# Autodesk Inventor assembly: mesoSPIM_excitation_path
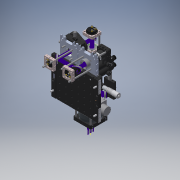
[picture p0: Inventor's stored thumbnail of the model, 180x180]
Saved by Autodesk Inventor 2016 (Build 200138000, 138)
## iProperties
Created: 2018-08-27
Part Number: mesoSPIM_excitation_path
Document SubType Name: Assembly
Designer: voigt
Author: voigt
## Documents named in this file (41)
- D:\Microscope_Design\CAD_Files\mesoSPIM_design_V5\mesoSPIM\excitation_path\mesoSPIM_excitation_path.iam
- D:\Microscope_Design\CAD_Files\mesoSPIM_design_V5\library\Thorlabs\large_area_translation_stages\tbb1515\TBB1515_M-Step.ipt
- D:\Microscope_Design\CAD_Files\mesoSPIM_design_V5\mesoSPIM\excitation_path\components\Galvomount-22mm-diameter-Thorlabs-Right.ipt
- D:\Microscope_Design\CAD_Files\mesoSPIM_design_V5\library\Thorlabs\posts\1_inch_posts\RS2P_M.ipt
- D:\Microscope_Design\CAD_Files\mesoSPIM_design_V5\library\Thorlabs\posts\1_5_inch_post_spacers\PS5M.ipt
- D:\Microscope_Design\CAD_Files\mesoSPIM_design_V5\library\Qioptiq\FLS40_rails\FLS40_150mm.ipt
- D:\Microscope_Design\CAD_Files\mesoSPIM_design_V5\library\Thorlabs\30mm_cage_system\base_plates\CPVM-60mm_Baseplate.ipt
- D:\Microscope_Design\CAD_Files\mesoSPIM_design_V5\library\Thorlabs\optics\AC254-075-A-ML-Step.ipt
- D:\Microscope_Design\CAD_Files\mesoSPIM_design_V5\mesoSPIM\optical_design\cad_export_v1\mesoSPIM_excitation_path_optics_V1.iam
- D:\Microscope_Design\CAD_Files\mesoSPIM_design_V5\library\Qioptiq\FLS40_carriers\FLS40_40mm_carrier.ipt
- D:\Microscope_Design\CAD_Files\mesoSPIM_design_V5\library\Qioptiq\microbench\Cube_30_with35hole.ipt
- D:\Microscope_Design\CAD_Files\mesoSPIM_design_V5\library\Qioptiq\microbench\Mounting_Plate_30.ipt
- D:\Microscope_Design\CAD_Files\mesoSPIM_design_V5\mesoSPIM\excitation_path\components\fold_mirror.iam
- D:\Microscope_Design\CAD_Files\mesoSPIM_design_V5\library\Qioptiq\FLS40_carriers\FLS40_20mm_carrier.ipt
- D:\Microscope_Design\CAD_Files\mesoSPIM_design_V5\library\Qioptiq\microbench\Mounting_Plate_35.ipt
- D:\Microscope_Design\CAD_Files\mesoSPIM_design_V5\library\Thorlabs\30mm_cage_system\cage_rods\ER3_CageRod.ipt
- D:\Microscope_Design\CAD_Files\Library_Files\Thorlabs\30mm_cage_system\rods\ER_CageRod.ipt
- D:\Microscope_Design\CAD_Files\mesoSPIM_design_V5\library\Thorlabs\30mm_cage_system\xy_mount\ST1XY-S_M-Step.ipt
- D:\Microscope_Design\CAD_Files\mesoSPIM_design_V5\library\Thorlabs\accessoires\SM1A39_Adapter_CmountExternal_SM1_External.ipt
- D:\Microscope_Design\CAD_Files\mesoSPIM_design_V5\library\Optotune\EL-16-40\EL-16-40-TC-C (133-193-03-R0-01).iam
- D:\Microscope_Design\CAD_Files\mesoSPIM_design_V5\library\Thorlabs\30mm_cage_system\cage_rods\ER1_CageRod.ipt
- D:\Microscope_Design\CAD_Files\mesoSPIM_design_V5\library\Thorlabs\30mm_cage_system\cage_rods\ER4_CageRod.ipt
- D:\Microscope_Design\CAD_Files\mesoSPIM_design_V5\library\Thorlabs\30mm_cage_system\cage_rods\ER2_CageRod.ipt
- D:\Microscope_Design\CAD_Files\mesoSPIM_design_V5\mesoSPIM\excitation_path\components\60mm-blank-cageplate-LCP03M-Nikon-MOD.ipt
- D:\Microscope_Design\CAD_Files\mesoSPIM_design_V5\library\Thorlabs\other\F-Mount-AdapterSM2NFM-Step.ipt
- D:\Microscope_Design\CAD_Files\mesoSPIM_design_V5\library\Nikon\50mm_1_4G_body_disassembled.ipt
- D:\Microscope_Design\CAD_Files\mesoSPIM_design_V5\library\Thorlabs\accessoires\SM1FCA-APC-Fiberadapter.ipt
- D:\Microscope_Design\CAD_Files\mesoSPIM_design_V5\library\Thorlabs\30mm_cage_system\cage_plates\SHCP025-Quarter-Inch-Shutter-Mount.ipt
- D:\Microscope_Design\CAD_Files\mesoSPIM_design_V5\library\Thorlabs\30mm_cage_system\cage_plates\CP02_M.ipt
- D:\Microscope_Design\CAD_Files\mesoSPIM_design_V5\library\Thorlabs\shutters\SHB025-Shutter.ipt
- D:\Microscope_Design\CAD_Files\mesoSPIM_design_V5\library\Thorlabs\30mm_cage_system\SM1_tubes\SM1L10.ipt
- D:\Microscope_Design\CAD_Files\mesoSPIM_design_V5\library\Thorlabs\30mm_cage_system\SM1_tubes\SM1V10.ipt
- D:\Microscope_Design\CAD_Files\mesoSPIM_design_V5\library\Qioptiq\microbench\35mm_lens_mount\35mm Lens Mount.ipt
- D:\Microscope_Design\CAD_Files\mesoSPIM_design_V5\library\Thorlabs\stages\XRN-B1_M-Micrometer-Baseplate.ipt
- D:\Microscope_Design\CAD_Files\mesoSPIM_design_V5\library\Thorlabs\stages\XRN25C_M-25mm-Micrometer-Stage-Simplified.ipt
- D:\Microscope_Design\CAD_Files\mesoSPIM_design_V5\library\Thorlabs\posts\post_mounts\PH75_M-Step.ipt
- D:\Microscope_Design\CAD_Files\mesoSPIM_design_V5\library\Thorlabs\posts\12_7_mm_posts\TR50M.ipt
- D:\Microscope_Design\CAD_Files\mesoSPIM_design_V5\library\Thorlabs\posts\12_7_mm_post_accessoires\RA180_M.ipt
- D:\Microscope_Design\CAD_Files\mesoSPIM_design_V5\library\Qioptiq\microbench\Microbench_Holder_30.iam
- D:\Microscope_Design\CAD_Files\mesoSPIM_design_V5\library\Thorlabs\posts\12_7_mm_posts\TR75M.ipt
- D:\Microscope_Design\CAD_Files\mesoSPIM_design_V5\library\Thorlabs\galvos\GVS411_M.ipt
## Components (62 placed, 39 different names)
1. TBB1515_M-Step:1 — Flush:1, Mate:1, Mate:2, Mate:3, Mate:4, Mate:5, Mate:6, Mate:7, Mate:8, Mate:10, Mate:18, Mate:19, Mate:20, Mate:22, Mate:96, Mate:97, Mate:98
2. Galvomount-22mm-diameter-Thorlabs-Right:1 — Mate:4, Mate:5, Mate:6, Flush:3, Mate:24, Mate:31, Mate:71, Mate:72, Flush:24, Angle:6, Mate:78, Angle:7, Mate:117, Mate:118, Angle:9
3. RS2P_M:1 — Mate:7, Mate:10, Mate:11, Mate:12
4. RS2P_M:2 — Mate:8, Mate:13, Mate:14, Mate:18
5. PS5M:1 — Mate:13, Mate:14, Mate:15, Mate:16
6. PS5M:2 — Mate:11, Mate:12, Mate:17
7. FLS40_150mm:1 — Mate:15, Flush:2, Flush:3, Mate:32, Mate:33, Flush:9, Mate:37, Mate:38
8. CPVM-60mm_Baseplate:1 — Mate:19, Flush:4, Mate:23, Mate:25, Mate:27, Mate:28, Mate:59, Flush:21, Mate:60, Flush:22, Mate:70, Mate:79, Mate:80, Flush:25, Flush:26, Mate:89, Mate:90, Mate:91
9. CPVM-60mm_Baseplate:2 — Mate:20, Mate:21, Mate:22, Flush:4, Mate:23, Mate:26, Mate:51, Angle:3, Mate:52, Mate:53, Mate:54, Mate:57, Flush:19, Mate:58, Flush:20, Mate:69
10. AC254-075-A-ML-Step:1 — Mate:27, Mate:28
11. mesoSPIM_excitation_path_optics_V1:1 [sub-assembly] — Mate:29, Mate:31
12. FLS40_40mm_carrier:1 — Mate:32, Mate:33, Mate:34, Flush:5, Flush:6, Flush:9
13. Cube_30_with35hole:1 — Mate:34, Flush:5, Flush:6, Flush:7, Mate:35, Flush:8, Mate:95, Flush:29, Flush:31
14. Mounting_Plate_30:1 — Flush:7, Mate:35, Flush:8, Mate:36, Flush:10, Angle:1
15. fold_mirror:1 [sub-assembly] — Mate:36, Flush:10, Angle:1
16. fold_mirror:2 [sub-assembly] — Mate:41, Angle:2, Mate:43
17. FLS40_20mm_carrier:1 — Mate:37, Mate:38, Mate:39, Flush:11, Flush:12
18. Mounting_Plate_35:1 — Mate:39, Flush:11, Flush:12, Flush:13, Flush:14, Mate:40, Flush:16, Flush:17, Flush:18
19. Mounting_Plate_35:2 — Flush:13, Flush:14, Mate:40, Mate:42, Flush:15, Mate:44, Mate:46, Mate:94, Flush:28
20. Mounting_Plate_30:2 — Flush:15, Flush:16, Angle:2, Mate:43, Mate:44, Mate:45
21. ER3_CageRod:1 — Mate:46, Flush:18
22. ER3_CageRod:2 — Mate:45, Flush:17
23. ST1XY-S_M-Step:1 — Mate:47, Mate:48, Mate:51, Angle:3, Mate:52, Mate:55, Mate:56
24. SM1A39_Adapter_CmountExternal_SM1_External:1 — Mate:47, Mate:48, Mate:49, Mate:50
25. EL-16-40-TC-C (133-193-03-R0-01):1 [sub-assembly] — Mate:49, Mate:50
26. ER1_CageRod:3 — Mate:53, Mate:55
27. ER1_CageRod:4 — Mate:54, Mate:56
28. ER4_CageRod:5 — Mate:58, Flush:20, Mate:64
29. ER4_CageRod:6 — Mate:57, Flush:19, Mate:63
30. ER4_CageRod:7 — Mate:59, Flush:21, Mate:62
31. ER4_CageRod:8 — Mate:60, Flush:22, Mate:61
32. Mounting_Plate_30:3 — Mate:63, Mate:64, Mate:67, Mate:68, Angle:4, Mate:69
33. Mounting_Plate_30:4 — Mate:61, Mate:62, Mate:65, Mate:66, Mate:70, Angle:5
34. fold_mirror:3 [sub-assembly] — Mate:67, Mate:68, Angle:4
35. fold_mirror:4 [sub-assembly] — Mate:65, Mate:66, Angle:5
36. ER2_CageRod:1 — Mate:71, Flush:23, Flush:24, Mate:77
37. ER2_CageRod:2 — Mate:72, Flush:23
38. 60mm-blank-cageplate-LCP03M-Nikon-MOD:1 — Mate:73, Mate:74, Mate:76, Mate:77, Angle:6, Mate:78
39. F-Mount-AdapterSM2NFM-Step:1 — Mate:73, Mate:74, Mate:75
40. 50mm_1_4G_body_disassembled:1 — Mate:75, Mate:76
41. ER3_CageRod:9 — Mate:79, Flush:26, Mate:81, Mate:83
42. ER3_CageRod:10 — Mate:80, Flush:25, Mate:82, Mate:84
43. SM1FCA-APC-Fiberadapter:1 — Mate:87, Mate:88
44. SHCP025-Quarter-Inch-Shutter-Mount:1 — Mate:81, Mate:82, Mate:85, Flush:27, Mate:86, Mate:89, Mate:93
45. CP02_M:1 — Mate:83, Mate:84, Mate:86, Mate:88
46. SHB025-Shutter:1 — Mate:85, Flush:27, Mate:87
47. SM1L10:1 — Mate:90, Mate:91, Mate:92
48. SM1V10:1 — Mate:92, Mate:93
49. 35mm Lens Mount:1 — Mate:94, Flush:28
50. 35mm Lens Mount:2 — Mate:95, Flush:29
51. XRN-B1_M-Micrometer-Baseplate:1 — Mate:96, Mate:97, Mate:98, Mate:99, Mate:100, Flush:30
52. XRN25C_M-25mm-Micrometer-Stage-Simplified:1 — Mate:99, Mate:100, Flush:30, Mate:101, Mate:102, Mate:103, Mate:104
53. PH75_M-Step:1 — Mate:101, Mate:104, Mate:109
54. PH75_M-Step:2 — Mate:102, Mate:103, Mate:110, Mate:116
55. TR50M:1 — Mate:105, Mate:106, Mate:109
56. TR50M:2 — Mate:107, Mate:108, Mate:110
57. RA180_M:1 — Mate:105, Mate:106, Mate:111
58. RA180_M:2 — Mate:107, Mate:108, Mate:114, Mate:116
59. Microbench_Holder_30:1 [sub-assembly] — Mate:112, Mate:113, Angle:7, Flush:31, Mate:115, Angle:8, Flush:32
60. TR75M:1 — Mate:111, Mate:112, Mate:113, Mate:114
61. fold_mirror:5 [sub-assembly] — Mate:115, Angle:8, Flush:32
62. GVS411_M:1 — Mate:117, Mate:118, Angle:9
## Relationships (158: Mate 117, Flush 32, Angle 9)
- Flush:1 (40 mm): TBB1515_M-Step:1
- Mate:1: TBB1515_M-Step:1
- Mate:2: TBB1515_M-Step:1
- Mate:3: TBB1515_M-Step:1
- Mate:4: TBB1515_M-Step:1 ↔ Galvomount-22mm-diameter-Thorlabs-Right:1
- Mate:5: TBB1515_M-Step:1 ↔ Galvomount-22mm-diameter-Thorlabs-Right:1
- Mate:6: TBB1515_M-Step:1 ↔ Galvomount-22mm-diameter-Thorlabs-Right:1
- Mate:7: TBB1515_M-Step:1 ↔ RS2P_M:1
- Mate:8: TBB1515_M-Step:1 ↔ RS2P_M:2
- Mate:10: TBB1515_M-Step:1 ↔ RS2P_M:1
- Mate:11: RS2P_M:1 ↔ PS5M:2
- Mate:12: RS2P_M:1 ↔ PS5M:2
- Mate:13: RS2P_M:2 ↔ PS5M:1
- Mate:14: RS2P_M:2 ↔ PS5M:1
- Mate:15: PS5M:1 ↔ FLS40_150mm:1
- Flush:2 (-20 mm): FLS40_150mm:1
- Mate:16: PS5M:1
- Mate:17: PS5M:2
- Flush:3: Galvomount-22mm-diameter-Thorlabs-Right:1 ↔ FLS40_150mm:1
- Mate:18: TBB1515_M-Step:1 ↔ RS2P_M:2
- Mate:19: TBB1515_M-Step:1 ↔ CPVM-60mm_Baseplate:1
- Mate:20: TBB1515_M-Step:1 ↔ CPVM-60mm_Baseplate:2
- Mate:21: CPVM-60mm_Baseplate:2
- Mate:22 (-2.98 mm): TBB1515_M-Step:1 ↔ CPVM-60mm_Baseplate:2
- Flush:4: CPVM-60mm_Baseplate:1 ↔ CPVM-60mm_Baseplate:2
- Mate:23 (75 mm): CPVM-60mm_Baseplate:1 ↔ CPVM-60mm_Baseplate:2
- Mate:24: Galvomount-22mm-diameter-Thorlabs-Right:1
- Mate:25: CPVM-60mm_Baseplate:1
- Mate:26: CPVM-60mm_Baseplate:2
- Mate:27: CPVM-60mm_Baseplate:1 ↔ AC254-075-A-ML-Step:1
- Mate:28: CPVM-60mm_Baseplate:1 ↔ AC254-075-A-ML-Step:1
- Mate:29: mesoSPIM_excitation_path_optics_V1:1
- Mate:30
- Mate:31: Galvomount-22mm-diameter-Thorlabs-Right:1 ↔ mesoSPIM_excitation_path_optics_V1:1
- Mate:32: FLS40_150mm:1 ↔ FLS40_40mm_carrier:1
- Mate:33: FLS40_150mm:1 ↔ FLS40_40mm_carrier:1
- Mate:34: FLS40_40mm_carrier:1 ↔ Cube_30_with35hole:1
- Flush:5: FLS40_40mm_carrier:1 ↔ Cube_30_with35hole:1
- Flush:6: FLS40_40mm_carrier:1 ↔ Cube_30_with35hole:1
- Flush:7: Cube_30_with35hole:1 ↔ Mounting_Plate_30:1
- Mate:35: Cube_30_with35hole:1 ↔ Mounting_Plate_30:1
- Flush:8: Cube_30_with35hole:1 ↔ Mounting_Plate_30:1
- Mate:36: Mounting_Plate_30:1 ↔ fold_mirror:1
- Flush:9: FLS40_150mm:1 ↔ FLS40_40mm_carrier:1
- Flush:10 (-3.3 mm): Mounting_Plate_30:1 ↔ fold_mirror:1
- Angle:1 (90 deg): Mounting_Plate_30:1 ↔ fold_mirror:1
- Mate:37: FLS40_150mm:1 ↔ FLS40_20mm_carrier:1
- Mate:38: FLS40_150mm:1 ↔ FLS40_20mm_carrier:1
- Mate:39: FLS40_20mm_carrier:1 ↔ Mounting_Plate_35:1
- Flush:11: FLS40_20mm_carrier:1 ↔ Mounting_Plate_35:1
- Flush:12: FLS40_20mm_carrier:1 ↔ Mounting_Plate_35:1
- Flush:13: Mounting_Plate_35:1 ↔ Mounting_Plate_35:2
- Flush:14: Mounting_Plate_35:1 ↔ Mounting_Plate_35:2
- Mate:40 (3 mm): Mounting_Plate_35:1 ↔ Mounting_Plate_35:2
- Mate:41: fold_mirror:2
- Mate:42: Mounting_Plate_35:2
- Flush:15: Mounting_Plate_35:2 ↔ Mounting_Plate_30:2
- Flush:16: Mounting_Plate_35:1 ↔ Mounting_Plate_30:2
- Angle:2 (90 deg): fold_mirror:2 ↔ Mounting_Plate_30:2
- Mate:43: fold_mirror:2 ↔ Mounting_Plate_30:2
- Mate:44 (43.5 mm): Mounting_Plate_35:2 ↔ Mounting_Plate_30:2
- Mate:45: Mounting_Plate_30:2 ↔ ER3_CageRod:2
- Flush:17: Mounting_Plate_35:1 ↔ ER3_CageRod:2
- Mate:46: Mounting_Plate_35:2 ↔ ER3_CageRod:1
- Flush:18: Mounting_Plate_35:1 ↔ ER3_CageRod:1
- Mate:47: ST1XY-S_M-Step:1 ↔ SM1A39_Adapter_CmountExternal_SM1_External:1
- Mate:48: ST1XY-S_M-Step:1 ↔ SM1A39_Adapter_CmountExternal_SM1_External:1
- Mate:49: SM1A39_Adapter_CmountExternal_SM1_External:1 ↔ EL-16-40-TC-C (133-193-03-R0-01):1
- Mate:50: SM1A39_Adapter_CmountExternal_SM1_External:1 ↔ EL-16-40-TC-C (133-193-03-R0-01):1
- Mate:51: CPVM-60mm_Baseplate:2 ↔ ST1XY-S_M-Step:1
- Angle:3 (90 deg): CPVM-60mm_Baseplate:2 ↔ ST1XY-S_M-Step:1
- Mate:52 (2 mm): CPVM-60mm_Baseplate:2 ↔ ST1XY-S_M-Step:1
- Mate:53: CPVM-60mm_Baseplate:2 ↔ ER1_CageRod:3
- Mate:54: CPVM-60mm_Baseplate:2 ↔ ER1_CageRod:4
- Mate:55: ST1XY-S_M-Step:1 ↔ ER1_CageRod:3
- Mate:56: ST1XY-S_M-Step:1 ↔ ER1_CageRod:4
- Mate:57: CPVM-60mm_Baseplate:2 ↔ ER4_CageRod:6
- Flush:19: CPVM-60mm_Baseplate:2 ↔ ER4_CageRod:6
- Mate:58: CPVM-60mm_Baseplate:2 ↔ ER4_CageRod:5
- Flush:20: CPVM-60mm_Baseplate:2 ↔ ER4_CageRod:5
- Mate:59: CPVM-60mm_Baseplate:1 ↔ ER4_CageRod:7
- Flush:21: CPVM-60mm_Baseplate:1 ↔ ER4_CageRod:7
- Mate:60: CPVM-60mm_Baseplate:1 ↔ ER4_CageRod:8
- Flush:22: CPVM-60mm_Baseplate:1 ↔ ER4_CageRod:8
- Mate:61: ER4_CageRod:8 ↔ Mounting_Plate_30:4
- Mate:62: ER4_CageRod:7 ↔ Mounting_Plate_30:4
- Mate:63: ER4_CageRod:6 ↔ Mounting_Plate_30:3
- Mate:64: ER4_CageRod:5 ↔ Mounting_Plate_30:3
- Mate:65: Mounting_Plate_30:4 ↔ fold_mirror:4
- Mate:66: Mounting_Plate_30:4 ↔ fold_mirror:4
- Mate:67: Mounting_Plate_30:3 ↔ fold_mirror:3
- Mate:68: Mounting_Plate_30:3 ↔ fold_mirror:3
- Angle:4 (0 deg): Mounting_Plate_30:3 ↔ fold_mirror:3
- Mate:69 (71 mm): CPVM-60mm_Baseplate:2 ↔ Mounting_Plate_30:3
- Mate:70 (71 mm): CPVM-60mm_Baseplate:1 ↔ Mounting_Plate_30:4
- Angle:5 (0 deg): Mounting_Plate_30:4 ↔ fold_mirror:4
- Mate:71: Galvomount-22mm-diameter-Thorlabs-Right:1 ↔ ER2_CageRod:1
- Mate:72: Galvomount-22mm-diameter-Thorlabs-Right:1 ↔ ER2_CageRod:2
- Flush:23: ER2_CageRod:1 ↔ ER2_CageRod:2
- Flush:24 (42 mm): Galvomount-22mm-diameter-Thorlabs-Right:1 ↔ ER2_CageRod:1
- Mate:73: 60mm-blank-cageplate-LCP03M-Nikon-MOD:1 ↔ F-Mount-AdapterSM2NFM-Step:1
- Mate:74: 60mm-blank-cageplate-LCP03M-Nikon-MOD:1 ↔ F-Mount-AdapterSM2NFM-Step:1
- Mate:75: F-Mount-AdapterSM2NFM-Step:1 ↔ 50mm_1_4G_body_disassembled:1
- Mate:76: 60mm-blank-cageplate-LCP03M-Nikon-MOD:1 ↔ 50mm_1_4G_body_disassembled:1
- Mate:77: ER2_CageRod:1 ↔ 60mm-blank-cageplate-LCP03M-Nikon-MOD:1
- Angle:6 (0 deg): Galvomount-22mm-diameter-Thorlabs-Right:1 ↔ 60mm-blank-cageplate-LCP03M-Nikon-MOD:1
- Mate:78 (30 mm): Galvomount-22mm-diameter-Thorlabs-Right:1 ↔ 60mm-blank-cageplate-LCP03M-Nikon-MOD:1
- Mate:79: CPVM-60mm_Baseplate:1 ↔ ER3_CageRod:9
- Mate:80: CPVM-60mm_Baseplate:1 ↔ ER3_CageRod:10
- Flush:25: CPVM-60mm_Baseplate:1 ↔ ER3_CageRod:10
- Flush:26: CPVM-60mm_Baseplate:1 ↔ ER3_CageRod:9
- Mate:81: ER3_CageRod:9 ↔ SHCP025-Quarter-Inch-Shutter-Mount:1
- Mate:82: ER3_CageRod:10 ↔ SHCP025-Quarter-Inch-Shutter-Mount:1
- Mate:83: ER3_CageRod:9 ↔ CP02_M:1
- Mate:84: ER3_CageRod:10 ↔ CP02_M:1
- Mate:85: SHCP025-Quarter-Inch-Shutter-Mount:1 ↔ SHB025-Shutter:1
- Flush:27: SHCP025-Quarter-Inch-Shutter-Mount:1 ↔ SHB025-Shutter:1
- Mate:86: SHCP025-Quarter-Inch-Shutter-Mount:1 ↔ CP02_M:1
- Mate:87: SM1FCA-APC-Fiberadapter:1 ↔ SHB025-Shutter:1
- Mate:88: SM1FCA-APC-Fiberadapter:1 ↔ CP02_M:1
- Mate:89 (48.9 mm): CPVM-60mm_Baseplate:1 ↔ SHCP025-Quarter-Inch-Shutter-Mount:1
- Mate:90: CPVM-60mm_Baseplate:1 ↔ SM1L10:1
- Mate:91: CPVM-60mm_Baseplate:1 ↔ SM1L10:1
- Mate:92: SM1L10:1 ↔ SM1V10:1
- Mate:93: SHCP025-Quarter-Inch-Shutter-Mount:1 ↔ SM1V10:1
- Mate:94: Mounting_Plate_35:2 ↔ 35mm Lens Mount:1
- Flush:28 (-0.6 mm): Mounting_Plate_35:2 ↔ 35mm Lens Mount:1
- Mate:95: Cube_30_with35hole:1 ↔ 35mm Lens Mount:2
- Flush:29 (8.45 mm): Cube_30_with35hole:1 ↔ 35mm Lens Mount:2
- Mate:96: TBB1515_M-Step:1 ↔ XRN-B1_M-Micrometer-Baseplate:1
- Mate:97: TBB1515_M-Step:1 ↔ XRN-B1_M-Micrometer-Baseplate:1
- Mate:98: TBB1515_M-Step:1 ↔ XRN-B1_M-Micrometer-Baseplate:1
- Mate:99: XRN-B1_M-Micrometer-Baseplate:1 ↔ XRN25C_M-25mm-Micrometer-Stage-Simplified:1
- Mate:100: XRN-B1_M-Micrometer-Baseplate:1 ↔ XRN25C_M-25mm-Micrometer-Stage-Simplified:1
- Flush:30: XRN-B1_M-Micrometer-Baseplate:1 ↔ XRN25C_M-25mm-Micrometer-Stage-Simplified:1
- Mate:101: XRN25C_M-25mm-Micrometer-Stage-Simplified:1 ↔ PH75_M-Step:1
- Mate:102: XRN25C_M-25mm-Micrometer-Stage-Simplified:1 ↔ PH75_M-Step:2
- Mate:103: XRN25C_M-25mm-Micrometer-Stage-Simplified:1 ↔ PH75_M-Step:2
- Mate:104: XRN25C_M-25mm-Micrometer-Stage-Simplified:1 ↔ PH75_M-Step:1
- Mate:105: TR50M:1 ↔ RA180_M:1
- Mate:106: TR50M:1 ↔ RA180_M:1
- Mate:107: TR50M:2 ↔ RA180_M:2
- Mate:108: TR50M:2 ↔ RA180_M:2
- Mate:109: PH75_M-Step:1 ↔ TR50M:1
- Mate:110: PH75_M-Step:2 ↔ TR50M:2
- Mate:111: RA180_M:1 ↔ TR75M:1
- Mate:112: Microbench_Holder_30:1 ↔ TR75M:1
- Mate:113: Microbench_Holder_30:1 ↔ TR75M:1
- Angle:7 (0 deg): Galvomount-22mm-diameter-Thorlabs-Right:1 ↔ Microbench_Holder_30:1
- Mate:114: RA180_M:2 ↔ TR75M:1
- Flush:31: Cube_30_with35hole:1 ↔ Microbench_Holder_30:1
- Mate:115: Microbench_Holder_30:1 ↔ fold_mirror:5
- Angle:8 (0 deg): Microbench_Holder_30:1 ↔ fold_mirror:5
- Mate:116: PH75_M-Step:2 ↔ RA180_M:2
- Flush:32 (4.4 mm): Microbench_Holder_30:1 ↔ fold_mirror:5
- Mate:117: Galvomount-22mm-diameter-Thorlabs-Right:1 ↔ GVS411_M:1
- Mate:118: Galvomount-22mm-diameter-Thorlabs-Right:1 ↔ GVS411_M:1
- Angle:9 (45 deg): Galvomount-22mm-diameter-Thorlabs-Right:1 ↔ GVS411_M:1
